# Autodesk Inventor assembly: Cross bar bracket + mounting design
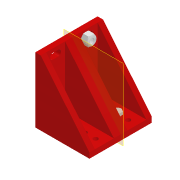
[picture p0: Inventor's stored thumbnail of the model, 180x180]
Saved by Autodesk Inventor 2020 (Build 240168000, 168)
## iProperties
Created: 2019-12-29
Part Number: Cross bar bracket + mounting design
Document SubType Name: Assembly
Designer: ball
Author: ball
## Documents named in this file (6)
- C:\FTC\FTC8863CAD\2019 Robot\Delivery\Cross bar bracket + mounting design.iam
- C:\FTC\FTC8863CAD\2019 Robot\Delivery\Cross bar bracket generic.ipt
- C:\FTC\FTC8863CAD\StepLibraries\Screws\M3 x 12 HEX HEAD CAP SCREW.ipt
- C:\FTC\FTC8863CAD\StepLibraries\Nuts\M4 NYLON-INSERT LOCKNUT.ipt
- C:\FTC\FTC8863CAD\StepLibraries\Washers\M4 FLAT WASHER.ipt
- C:\FTC\FTC8863CAD\StepLibraries\Screws\M4 x 12 SOCKET HEAD CAP SCREW.ipt
## Components (7 placed, 5 different names)
1. Cross bar bracket generic:1 — Mate:1, Mate:2, Mate:3, Mate:4, Mate:7, Mate:8, Mate:9, Mate:10, Mate:11, Mate:12
2. M3 x 12 HEX HEAD CAP SCREW:2 — Mate:1, Mate:2
3. M4 NYLON-INSERT LOCKNUT:1 — Mate:3, Mate:4
4. M4 FLAT WASHER:1 — Mate:7, Mate:8
5. M3 x 12 HEX HEAD CAP SCREW:3 — Mate:9, Mate:10
6. M4 FLAT WASHER:2 — Mate:11, Mate:12, Mate:13, Mate:14
7. M4 x 12 SOCKET HEAD CAP SCREW:1 — Mate:13, Mate:14
## Relationships (12: Mate 12)
- Mate:1: Cross bar bracket generic:1 ↔ M3 x 12 HEX HEAD CAP SCREW:2
- Mate:2: Cross bar bracket generic:1 ↔ M3 x 12 HEX HEAD CAP SCREW:2
- Mate:3: Cross bar bracket generic:1 ↔ M4 NYLON-INSERT LOCKNUT:1
- Mate:4: Cross bar bracket generic:1 ↔ M4 NYLON-INSERT LOCKNUT:1
- Mate:7: Cross bar bracket generic:1 ↔ M4 FLAT WASHER:1
- Mate:8: Cross bar bracket generic:1 ↔ M4 FLAT WASHER:1
- Mate:9: Cross bar bracket generic:1 ↔ M3 x 12 HEX HEAD CAP SCREW:3
- Mate:10: Cross bar bracket generic:1 ↔ M3 x 12 HEX HEAD CAP SCREW:3
- Mate:11: Cross bar bracket generic:1 ↔ M4 FLAT WASHER:2
- Mate:12: Cross bar bracket generic:1 ↔ M4 FLAT WASHER:2
- Mate:13: M4 FLAT WASHER:2 ↔ M4 x 12 SOCKET HEAD CAP SCREW:1
- Mate:14: M4 FLAT WASHER:2 ↔ M4 x 12 SOCKET HEAD CAP SCREW:1
